# Autodesk Inventor assembly: baseAssem
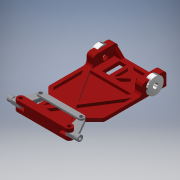
[picture p0: Inventor's stored thumbnail of the model, 180x180]
Saved by Autodesk Inventor 2018 (Build 220112000, 112)
## iProperties
Created: 2018-07-12
Part Number: baseAssem
Document SubType Name: Assembly
Designer: Cole Tucker
Author: Cole Tucker
## Documents named in this file (5)
- C:\Users\Cole Tucker\OneDrive\FRC-mxpProject\Cad\TestCar\baseAssem.iam
- C:\Users\Cole Tucker\OneDrive\FRC-mxpProject\Cad\TestCar\frame.ipt
- C:\Users\Cole Tucker\OneDrive\FRC-mxpProject\Cad\TestCar\bearing.ipt
- C:\Users\Cole Tucker\OneDrive\FRC-mxpProject\Cad\TestCar\StteringArm.ipt
- C:\Users\Cole Tucker\OneDrive\FRC-mxpProject\Cad\TestCar\linkage.ipt
## Components (6 placed, 4 different names)
1. frame:1 — Mate:1, Mate:2, Mate:3, Mate:4, Mate:5, Mate:6, Mate:7, Mate:8
2. bearing:1 — Mate:1, Mate:2
3. bearing:2 — Mate:3, Mate:4
4. StteringArm:1 — Mate:7, Mate:8, Mate:9, Mate:10
5. StteringArm:2 — Mate:5, Mate:6, Mate:11
6. linkage:1 — Mate:9, Mate:10, Mate:11
## Relationships (11: Mate 11)
- Mate:1: frame:1 ↔ bearing:1
- Mate:2: frame:1 ↔ bearing:1
- Mate:3: frame:1 ↔ bearing:2
- Mate:4: frame:1 ↔ bearing:2
- Mate:5: frame:1 ↔ StteringArm:2
- Mate:6: frame:1 ↔ StteringArm:2
- Mate:7: frame:1 ↔ StteringArm:1
- Mate:8: frame:1 ↔ StteringArm:1
- Mate:9: StteringArm:1 ↔ linkage:1
- Mate:10: StteringArm:1 ↔ linkage:1
- Mate:11: StteringArm:2 ↔ linkage:1
